# Autodesk Inventor assembly: Weapon (Motor-Side Pulley)
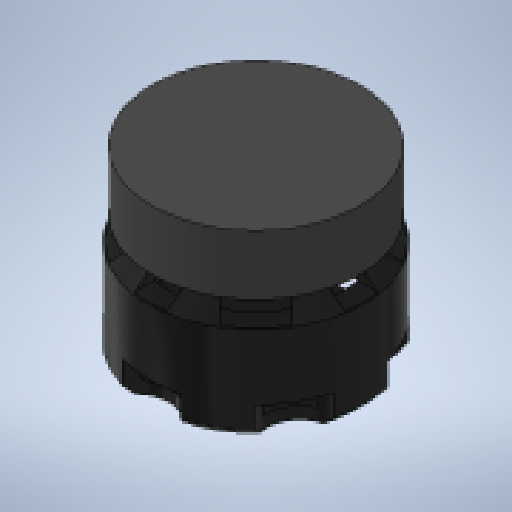
[picture p0: Inventor's stored thumbnail of the model, 512x512]
Saved by Autodesk Inventor 2023.1 (Build 271208000, 208)
## iProperties
Created: 2022-05-21
Part Number: Weapon (Motor-Side Pulley)
Document SubType Name: Assembly
Designer: Nathan Cai
Mass: 100 g
Surface Area: 105.713 cm^2
Volume: 11.2621 cm^3
Density: 8.87931 g/cm^3
Author: Nathan Cai
## Documents named in this file (3)
- E:\Documents\Inventor\0.3rd Lawette - V3.4\Horizontal Weapon Assembly (Type U)\Weapon (Motor-Side Pulley).iam
- E:\Documents\Inventor\0.3rd Lawette - V3.4\Horizontal Weapon Assembly (Type U)\AeroSky_MC4822-390KV.ipt
- E:\Documents\Inventor\0.3rd Lawette - V3.4\Horizontal Weapon Assembly (Type U)\Placeholder (Gear - M).ipt
## Components (2 placed, 2 different names)
1. AeroSky_MC4822-390KV:1 — Mate:1, Mate:2
2. Placeholder (Gear - M):1 — Mate:1, Mate:2
## Relationships (2: Mate 2)
- Mate:1: AeroSky_MC4822-390KV:1 ↔ Placeholder (Gear - M):1
- Mate:2 (-38.1 mm): AeroSky_MC4822-390KV:1 ↔ Placeholder (Gear - M):1
